# Autodesk Inventor assembly: assembly
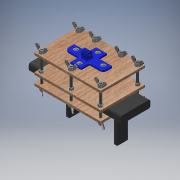
[picture p0: Inventor's stored thumbnail of the model, 180x180]
Saved by Autodesk Inventor 2018 (Build 220112000, 112)
## iProperties
Created: 2019-06-17
Part Number: assembly
Document SubType Name: Assembly
Designer: ZEUSLAP
Author: ZEUSLAP
## Documents named in this file (12)
- C:\Users\ZEUSLAP\YandexDisk\Inventor\balcony-railing-clamp\assembly.iam
- C:\Users\ZEUSLAP\YandexDisk\Inventor\balcony-railing-clamp\models\railing_fragment.ipt
- C:\Users\ZEUSLAP\YandexDisk\Inventor\balcony-railing-clamp\models\plywood\top.ipt
- C:\Users\ZEUSLAP\YandexDisk\Inventor\balcony-railing-clamp\models\plywood\bottom.ipt
- C:\Users\ZEUSLAP\YandexDisk\Inventor\balcony-railing-clamp\models\Threaded rod M6.ipt
- C:\Users\ZEUSLAP\Documents\Inventor\Content Center Files\R2018\en-US\ANSI B 18.2.4.1 M(1)\ANSI B 18.2.4.1 M - M6 x 1Style 2.ipt
- C:\Users\ZEUSLAP\Documents\Inventor\Content Center Files\R2018\en-US\DIN 315\DIN 315 - M6.ipt
- C:\Users\ZEUSLAP\YandexDisk\Inventor\balcony-railing-clamp\models\printed\action_cam_connector.ipt
- C:\Users\ZEUSLAP\YandexDisk\Inventor\balcony-railing-clamp\models\plywood\connector_mount.ipt
- C:\Users\ZEUSLAP\Documents\Inventor\Content Center Files\R2018\en-US\ISO 7093 A\ISO 7093 A - ST 4 - 140 HV .ipt
- C:\Users\ZEUSLAP\Documents\Inventor\Content Center Files\R2018\en-US\ANSI B 18.2.4.1 M(1)\ANSI B 18.2.4.1 M - M4 x 0.7Style 2.ipt
- C:\Users\ZEUSLAP\Documents\Inventor\Content Center Files\R2018\en-US\DIN 7985 (H)\DIN 7985 (H) - M4x16-H.ipt
## Components (52 placed, 11 different names)
1. railing_fragment:1 — Mate:1, Flush:1, Flush:2, Mate:2, Mate:78
2. top:1 — Mate:1, Flush:1, Flush:2, Flush:3, Flush:4, Mate:3, Mate:7, Mate:10, Mate:11, Mate:12, Mate:13, Mate:14, Mate:15, Mate:31, Mate:33, Mate:35, Mate:37, Mate:39, Mate:41, Mate:74
3. bottom:1 — Mate:2, Flush:3, Flush:4, Mate:9, Flush:11, Mate:19, Mate:21, Mate:23, Mate:25, Mate:27, Mate:29
4. Threaded rod M6:1 — Mate:3, Mate:6, Mate:8, Flush:5, Flush:11, Mate:71, Mate:87, Mate:109
5. Threaded rod M6:2 — Mate:10, Flush:9, Mate:26, Mate:40, Mate:93, Mate:97
6. Threaded rod M6:3 — Mate:12, Flush:10, Mate:22, Mate:36, Mate:95, Mate:101
7. Threaded rod M6:4 — Mate:11, Flush:8, Flush:9, Mate:24, Mate:38, Mate:91, Mate:99
8. Threaded rod M6:5 — Mate:15, Flush:5, Flush:6, Mate:18, Mate:30, Mate:85, Mate:107
9. Threaded rod M6:6 — Mate:13, Flush:7, Flush:8, Flush:10, Mate:28, Mate:34, Mate:73, Mate:89, Mate:103
10. Threaded rod M6:7 — Mate:14, Flush:6, Flush:7, Mate:20, Mate:32, Mate:72, Mate:83, Mate:105
11. Hex Nut Metric M6 x 1:3 — Mate:26, Mate:27
12. Hex Nut Metric M6 x 1:4 — Mate:28, Mate:29
13. DIN 315 M6:1 — Mate:8, Mate:9
14. DIN 315 M6:2 — Mate:18, Mate:19
15. DIN 315 M6:3 — Mate:20, Mate:21
16. DIN 315 M6:4 — Mate:22, Mate:23
17. DIN 315 M6:5 — Mate:24, Mate:25
18. Hex Nut Metric M6 x 1:2 — Mate:6, Mate:7
19. Hex Nut Metric M6 x 1:5 — Mate:30, Mate:31
20. Hex Nut Metric M6 x 1:6 — Mate:32, Mate:33
21. Hex Nut Metric M6 x 1:7 — Mate:34, Mate:35
22. Hex Nut Metric M6 x 1:8 — Mate:36, Mate:37
23. Hex Nut Metric M6 x 1:9 — Mate:38, Mate:39
24. Hex Nut Metric M6 x 1:10 — Mate:40, Mate:41
25. action_cam_connector:1 — Mate:80, Mate:81, Mate:82, Insert:1, Insert:2, Insert:3, Insert:4
26. connector_mount:1 — Mate:71, Mate:72, Mate:73, Mate:74, Mate:79, Mate:80, Mate:81, Mate:82, Mate:84, Mate:86, Mate:88, Mate:90, Mate:92, Mate:94, Mate:96, Mate:98, Mate:100, Mate:102, Mate:104, Mate:106, Mate:108, Mate:110, Mate:112, Mate:114, Mate:116, Mate:118
27. Hex Nut Metric M6 x 1:11 — Mate:83, Mate:84
28. Hex Nut Metric M6 x 1:12 — Mate:85, Mate:86
29. Hex Nut Metric M6 x 1:13 — Mate:87, Mate:88
30. Hex Nut Metric M6 x 1:14 — Mate:89, Mate:90
31. Hex Nut Metric M6 x 1:15 — Mate:91, Mate:92
32. Hex Nut Metric M6 x 1:16 — Mate:93, Mate:94
33. Hex Nut Metric M6 x 1:17 — Mate:95, Mate:96
34. DIN 315 M6:6 — Mate:97, Mate:98
35. DIN 315 M6:7 — Mate:99, Mate:100
36. DIN 315 M6:8 — Mate:101, Mate:102
37. DIN 315 M6:9 — Mate:103, Mate:104
38. DIN 315 M6:10 — Mate:105, Mate:106
39. DIN 315 M6:11 — Mate:107, Mate:108
40. DIN 315 M6:12 — Mate:109, Mate:110
41. ISO 7093 A ST 4 - 140 HV - A:1 — Insert:1, Insert:9
42. ISO 7093 A ST 4 - 140 HV - A:2 — Insert:2, Insert:6
43. ISO 7093 A ST 4 - 140 HV - A:3 — Insert:3, Insert:8
44. ISO 7093 A ST 4 - 140 HV - A:4 — Insert:4, Insert:7
45. DIN 7985 (H) M4x16-H:1 — Insert:6, Mate:113
46. DIN 7985 (H) M4x16-H:2 — Insert:7, Mate:111
47. DIN 7985 (H) M4x16-H:3 — Insert:8, Mate:115
48. DIN 7985 (H) M4x16-H:4 — Insert:9, Mate:117
49. Hex Nut Metric M4 x 0.7:1 — Mate:111, Mate:112
50. Hex Nut Metric M4 x 0.7:2 — Mate:113, Mate:114
51. Hex Nut Metric M4 x 0.7:3 — Mate:115, Mate:116
52. Hex Nut Metric M4 x 0.7:4 — Mate:117, Mate:118
## Relationships (101: Mate 82, Flush 11, Insert 8)
- Mate:1: railing_fragment:1 ↔ top:1
- Flush:1 (20 mm): railing_fragment:1 ↔ top:1
- Flush:2 (-20 mm): railing_fragment:1 ↔ top:1
- Mate:2: railing_fragment:1 ↔ bottom:1
- Flush:3: top:1 ↔ bottom:1
- Flush:4: top:1 ↔ bottom:1
- Mate:3: top:1 ↔ Threaded rod M6:1
- Mate:6: Threaded rod M6:1 ↔ Hex Nut Metric M6 x 1:2
- Mate:7: top:1 ↔ Hex Nut Metric M6 x 1:2
- Mate:8: Threaded rod M6:1 ↔ DIN 315 M6:1
- Mate:9: bottom:1 ↔ DIN 315 M6:1
- Mate:10: top:1 ↔ Threaded rod M6:2
- Mate:11: top:1 ↔ Threaded rod M6:4
- Mate:12: top:1 ↔ Threaded rod M6:3
- Mate:13: top:1 ↔ Threaded rod M6:6
- Mate:14: top:1 ↔ Threaded rod M6:7
- Mate:15: top:1 ↔ Threaded rod M6:5
- Flush:5: Threaded rod M6:1 ↔ Threaded rod M6:5
- Flush:6: Threaded rod M6:5 ↔ Threaded rod M6:7
- Flush:7: Threaded rod M6:6 ↔ Threaded rod M6:7
- Flush:8: Threaded rod M6:4 ↔ Threaded rod M6:6
- Flush:9: Threaded rod M6:2 ↔ Threaded rod M6:4
- Flush:10: Threaded rod M6:3 ↔ Threaded rod M6:6
- Flush:11 (-12 mm): bottom:1 ↔ Threaded rod M6:1
- Mate:18: Threaded rod M6:5 ↔ DIN 315 M6:2
- Mate:19: bottom:1 ↔ DIN 315 M6:2
- Mate:20: Threaded rod M6:7 ↔ DIN 315 M6:3
- Mate:21: bottom:1 ↔ DIN 315 M6:3
- Mate:22: Threaded rod M6:3 ↔ DIN 315 M6:4
- Mate:23: bottom:1 ↔ DIN 315 M6:4
- Mate:24: Threaded rod M6:4 ↔ DIN 315 M6:5
- Mate:25: bottom:1 ↔ DIN 315 M6:5
- Mate:26: Threaded rod M6:2 ↔ Hex Nut Metric M6 x 1:3
- Mate:27: bottom:1 ↔ Hex Nut Metric M6 x 1:3
- Mate:28: Threaded rod M6:6 ↔ Hex Nut Metric M6 x 1:4
- Mate:29: bottom:1 ↔ Hex Nut Metric M6 x 1:4
- Mate:30: Threaded rod M6:5 ↔ Hex Nut Metric M6 x 1:5
- Mate:31: top:1 ↔ Hex Nut Metric M6 x 1:5
- Mate:32: Threaded rod M6:7 ↔ Hex Nut Metric M6 x 1:6
- Mate:33: top:1 ↔ Hex Nut Metric M6 x 1:6
- Mate:34: Threaded rod M6:6 ↔ Hex Nut Metric M6 x 1:7
- Mate:35: top:1 ↔ Hex Nut Metric M6 x 1:7
- Mate:36: Threaded rod M6:3 ↔ Hex Nut Metric M6 x 1:8
- Mate:37: top:1 ↔ Hex Nut Metric M6 x 1:8
- Mate:38: Threaded rod M6:4 ↔ Hex Nut Metric M6 x 1:9
- Mate:39: top:1 ↔ Hex Nut Metric M6 x 1:9
- Mate:40: Threaded rod M6:2 ↔ Hex Nut Metric M6 x 1:10
- Mate:41: top:1 ↔ Hex Nut Metric M6 x 1:10
- Mate:71: Threaded rod M6:1 ↔ connector_mount:1
- Mate:72: Threaded rod M6:7 ↔ connector_mount:1
- Mate:73: Threaded rod M6:6 ↔ connector_mount:1
- Mate:74 (40 mm): top:1 ↔ connector_mount:1
- Mate:78: railing_fragment:1
- Mate:79: connector_mount:1
- Mate:80: action_cam_connector:1 ↔ connector_mount:1
- Mate:81: action_cam_connector:1 ↔ connector_mount:1
- Mate:82: action_cam_connector:1 ↔ connector_mount:1
- Mate:83: Threaded rod M6:7 ↔ Hex Nut Metric M6 x 1:11
- Mate:84: connector_mount:1 ↔ Hex Nut Metric M6 x 1:11
- Mate:85: Threaded rod M6:5 ↔ Hex Nut Metric M6 x 1:12
- Mate:86: connector_mount:1 ↔ Hex Nut Metric M6 x 1:12
- Mate:87: Threaded rod M6:1 ↔ Hex Nut Metric M6 x 1:13
- Mate:88: connector_mount:1 ↔ Hex Nut Metric M6 x 1:13
- Mate:89: Threaded rod M6:6 ↔ Hex Nut Metric M6 x 1:14
- Mate:90: connector_mount:1 ↔ Hex Nut Metric M6 x 1:14
- Mate:91: Threaded rod M6:4 ↔ Hex Nut Metric M6 x 1:15
- Mate:92: connector_mount:1 ↔ Hex Nut Metric M6 x 1:15
- Mate:93: Threaded rod M6:2 ↔ Hex Nut Metric M6 x 1:16
- Mate:94: connector_mount:1 ↔ Hex Nut Metric M6 x 1:16
- Mate:95: Threaded rod M6:3 ↔ Hex Nut Metric M6 x 1:17
- Mate:96: connector_mount:1 ↔ Hex Nut Metric M6 x 1:17
- Mate:97: Threaded rod M6:2 ↔ DIN 315 M6:6
- Mate:98: connector_mount:1 ↔ DIN 315 M6:6
- Mate:99: Threaded rod M6:4 ↔ DIN 315 M6:7
- Mate:100: connector_mount:1 ↔ DIN 315 M6:7
- Mate:101: Threaded rod M6:3 ↔ DIN 315 M6:8
- Mate:102: connector_mount:1 ↔ DIN 315 M6:8
- Mate:103: Threaded rod M6:6 ↔ DIN 315 M6:9
- Mate:104: connector_mount:1 ↔ DIN 315 M6:9
- Mate:105: Threaded rod M6:7 ↔ DIN 315 M6:10
- Mate:106: connector_mount:1 ↔ DIN 315 M6:10
- Mate:107: Threaded rod M6:5 ↔ DIN 315 M6:11
- Mate:108: connector_mount:1 ↔ DIN 315 M6:11
- Mate:109: Threaded rod M6:1 ↔ DIN 315 M6:12
- Mate:110: connector_mount:1 ↔ DIN 315 M6:12
- Insert:1: action_cam_connector:1 ↔ ISO 7093 A ST 4 - 140 HV - A:1
- Insert:2: action_cam_connector:1 ↔ ISO 7093 A ST 4 - 140 HV - A:2
- Insert:3: action_cam_connector:1 ↔ ISO 7093 A ST 4 - 140 HV - A:3
- Insert:4: action_cam_connector:1 ↔ ISO 7093 A ST 4 - 140 HV - A:4
- Insert:6: ISO 7093 A ST 4 - 140 HV - A:2 ↔ DIN 7985 (H) M4x16-H:1
- Insert:7: ISO 7093 A ST 4 - 140 HV - A:4 ↔ DIN 7985 (H) M4x16-H:2
- Insert:8: ISO 7093 A ST 4 - 140 HV - A:3 ↔ DIN 7985 (H) M4x16-H:3
- Mate:111: DIN 7985 (H) M4x16-H:2 ↔ Hex Nut Metric M4 x 0.7:1
- Mate:112: connector_mount:1 ↔ Hex Nut Metric M4 x 0.7:1
- Mate:113: DIN 7985 (H) M4x16-H:1 ↔ Hex Nut Metric M4 x 0.7:2
- Mate:114: connector_mount:1 ↔ Hex Nut Metric M4 x 0.7:2
- Mate:115: DIN 7985 (H) M4x16-H:3 ↔ Hex Nut Metric M4 x 0.7:3
- Mate:116: connector_mount:1 ↔ Hex Nut Metric M4 x 0.7:3
- Insert:9: ISO 7093 A ST 4 - 140 HV - A:1 ↔ DIN 7985 (H) M4x16-H:4
- Mate:117: DIN 7985 (H) M4x16-H:4 ↔ Hex Nut Metric M4 x 0.7:4
- Mate:118: connector_mount:1 ↔ Hex Nut Metric M4 x 0.7:4
